# Autodesk Inventor assembly: Camera
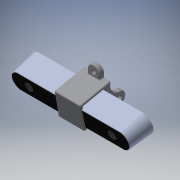
[picture p0: Inventor's stored thumbnail of the model, 180x180]
Saved by Autodesk Inventor 2017 SP1 (Build 210196100, 196)
## iProperties
Created: 2016-09-29
Part Number: Camera
Document SubType Name: Assembly
Designer: Haden
Author: Haden
## Documents named in this file (3)
- C:\Users\Haden\Desktop\Charlie-CAD-Model\Robot Model\Camera\Camera.iam
- C:\Users\Haden\Desktop\Charlie-CAD-Model\Robot Model\Camera\ZED-camera.iam
- C:\Users\Haden\Desktop\Charlie-CAD-Model\Robot Model\Camera\Camera Mount.ipt
## Components (2 placed, 2 different names)
1. Camera Mount:1 — Insert:1, Rotation:1
2. ZED-camera:1 [sub-assembly] — Insert:1, Rotation:1
## Relationships (2: Insert 1, RelateRotation 1)
- Insert:1: Camera Mount:1 ↔ ZED-camera:1
- Rotation:1 [RelateRotation] (1 ul): Camera Mount:1 ↔ ZED-camera:1
